# Autodesk Inventor assembly: ShaftAssembly
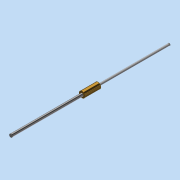
[picture p0: Inventor's stored thumbnail of the model, 180x180]
Saved by Autodesk Inventor 2017 (Build 210142000, 142)
## iProperties
Created: 2017-04-13
Part Number: ShaftAssembly
Document SubType Name: Assembly
Designer: techn
Mass: 38.5837 g
Surface Area: 44.2181 cm^2
Volume: 4.75098 cm^3
Density: 8.12122 g/cm^3
Author: techn
## Documents named in this file (4)
- D:\OneDrive\Documents\Other Projects\Submarine\CAD\test\ShaftAssembly.iam
- D:\OneDrive\Documents\Other Projects\Submarine\CAD\test\Coupler.ipt
- D:\OneDrive\Documents\Other Projects\Submarine\CAD\test\Shaft.ipt
- D:\OneDrive\Documents\Other Projects\Submarine\CAD\test\Shaft2.ipt
## Components (3 placed, 3 different names)
1. Coupler:1 — Mate:1, Mate:2, Mate:3
2. Shaft:1 — Mate:1, Mate:2, Mate:4
3. Shaft2:1 — Mate:3, Mate:4
## Relationships (4: Mate 4)
- Mate:1: Coupler:1 ↔ Shaft:1
- Mate:2: Coupler:1 ↔ Shaft:1
- Mate:3: Coupler:1 ↔ Shaft2:1
- Mate:4: Shaft:1 ↔ Shaft2:1
